# Autodesk Inventor assembly: LS Conveyor Axle
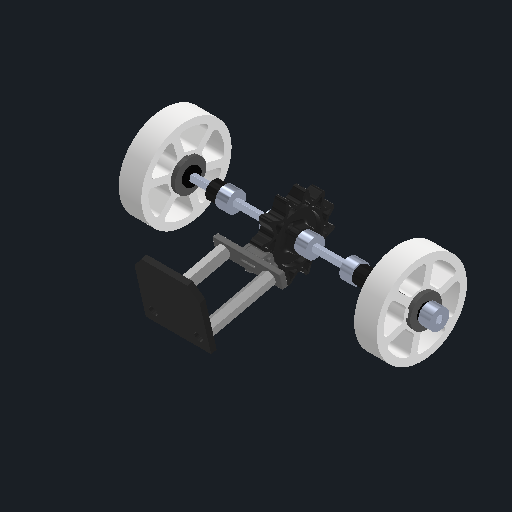
[picture p0: Inventor's stored thumbnail of the model, 512x512]
Saved by Autodesk Inventor 2025 (Build 290162000, 162)
## iProperties
Created: 2024-12-19
Part Number: LS Conveyor Axle
Document SubType Name: Assembly
Designer: Juan
Author: Juan
## Documents named in this file (14)
- C:\Users\Juan\Documents\GitHub\ATUM-VRC-High-Stakes-CAD\Protobot\LS Conveyor Axle.iam
- C:\Users\Juan\Documents\GitHub\ATUM-VRC-High-Stakes-CAD\VEX-CAD-Inventor\Motion\Sprockets\9P Sprocket\9P 12T Sprocket, Square.iam
- C:\Users\Juan\Documents\GitHub\ATUM-VRC-High-Stakes-CAD\VEX-CAD-Inventor\Motion\Sprockets\9P Sprocket.iam
- C:\Users\Juan\Documents\GitHub\ATUM-VRC-High-Stakes-CAD\VEX-CAD-Inventor\Motion\Chain 9P\Chain Attachment Link.ipt
- C:\Users\Juan\Documents\GitHub\ATUM-VRC-High-Stakes-CAD\Hook.ipt
- C:\Users\Juan\Documents\GitHub\ATUM-VRC-High-Stakes-CAD\VEX-CAD-Inventor\Structure\Standoff\Standoff 1.50.ipt
- C:\Users\Juan\Documents\GitHub\ATUM-VRC-High-Stakes-CAD\VEX-CAD-Inventor\Structure\Standoff.ipt
- C:\Users\Juan\Documents\GitHub\ATUM-VRC-High-Stakes-CAD\VEX-CAD-Inventor\Motion\Shaft LS\Shaft LS\Shaft LS 6.5.ipt
- C:\Users\Juan\Documents\GitHub\ATUM-VRC-High-Stakes-CAD\VEX-CAD-Inventor\Motion\Shaft LS\Shaft LS.ipt
- C:\Users\Juan\Documents\GitHub\ATUM-VRC-High-Stakes-CAD\VEX-CAD-Inventor\Motion\Shaft LS\Shaft Collar Metal\Shaft Collar No Screw.ipt
- C:\Users\Juan\Documents\GitHub\ATUM-VRC-High-Stakes-CAD\VEX-CAD-Inventor\Motion\Spacers\Spacer Nylon .375 OD\NSpacer .375 OD x .250.ipt
- C:\Users\Juan\Documents\GitHub\ATUM-VRC-High-Stakes-CAD\VEX-CAD-Inventor\Motion\Spacers\Spacer Nylon .375 OD.ipt
- C:\Users\Juan\Documents\GitHub\ATUM-VRC-High-Stakes-CAD\VEX-CAD-Inventor\Motion\Insert Square.ipt
- C:\Users\Juan\Documents\GitHub\ATUM-VRC-High-Stakes-CAD\Protobot\2.0 Flex Wheel with Insert.iam
## Components (20 placed, 9 different names)
1. 9P 12T Sprocket, Square:1 [sub-assembly]
2. Chain Attachment Link:1
3. Hook:1
4. Standoff 1.50:1
5. Standoff 1.50:2
6. Shaft LS 6.5:1
7. Shaft Collar No Screw:1
8. Shaft Collar No Screw:2
9. NSpacer .375 OD x .250:1
10. NSpacer .375 OD x .250:2
11. Shaft Collar No Screw:3
12. Shaft Collar No Screw:4
13. Insert Square:1
14. Insert Square:2
15. Insert Square:3
16. Insert Square:4
17. Shaft Collar No Screw:5
18. Shaft Collar No Screw:6
19. 2.0 Flex Wheel with Insert:1 [sub-assembly]
20. 2.0 Flex Wheel with Insert:2 [sub-assembly]
## Relationships (45: Mate 37, Angle 6, Flush 2)
- [Mate]: 9P 12T Sprocket, Square:1 ↔ Chain Attachment Link:1
- [Mate] (-2.54 mm): 9P 12T Sprocket, Square:1 ↔ Chain Attachment Link:1
- [Mate]: Chain Attachment Link:1 ↔ Standoff 1.50:1
- [Mate]: Chain Attachment Link:1 ↔ Standoff 1.50:2
- [Mate]: Chain Attachment Link:1 ↔ Standoff 1.50:2
- [Mate] (0.1524 mm): 9P 12T Sprocket, Square:1 ↔ Chain Attachment Link:1
- [Mate]: Chain Attachment Link:1 ↔ Standoff 1.50:1
- [Mate]: Hook:1 ↔ Standoff 1.50:1
- [Mate]: Hook:1 ↔ Standoff 1.50:2
- [Mate]: Hook:1 ↔ Standoff 1.50:2
- [Mate]: 9P 12T Sprocket, Square:1 ↔ Shaft LS 6.5:1
- [Mate]: 9P 12T Sprocket, Square:1 ↔ Shaft LS 6.5:1
- [Mate]: 9P 12T Sprocket, Square:1 ↔ Shaft Collar No Screw:1
- [Mate]: 9P 12T Sprocket, Square:1 ↔ Shaft Collar No Screw:2
- [Mate]: NSpacer .375 OD x .250:1 ↔ Shaft Collar No Screw:3
- [Mate]: NSpacer .375 OD x .250:1 ↔ Shaft Collar No Screw:3
- [Angle] (0 deg): Shaft LS 6.5:1 ↔ Shaft Collar No Screw:1
- [Angle] (0 deg): Shaft LS 6.5:1 ↔ Shaft Collar No Screw:2
- [Angle] (0 deg): Shaft LS 6.5:1 ↔ Shaft Collar No Screw:3
- [Mate]: NSpacer .375 OD x .250:2 ↔ Shaft Collar No Screw:4
- [Angle] (0 deg): Shaft LS 6.5:1 ↔ Shaft Collar No Screw:4
- [Mate]: Insert Square:1 ↔ 2.0 Flex Wheel with Insert:1
- [Mate]: Insert Square:1 ↔ 2.0 Flex Wheel with Insert:1
- [Mate]: Insert Square:2 ↔ 2.0 Flex Wheel with Insert:1
- [Mate]: Insert Square:2 ↔ 2.0 Flex Wheel with Insert:1
- [Mate]: Insert Square:3 ↔ 2.0 Flex Wheel with Insert:2
- [Mate]: Insert Square:3 ↔ 2.0 Flex Wheel with Insert:2
- [Mate]: Insert Square:4 ↔ 2.0 Flex Wheel with Insert:2
- [Mate]: Insert Square:4 ↔ 2.0 Flex Wheel with Insert:2
- [Mate]: Insert Square:3 ↔ 2.0 Flex Wheel with Insert:2
- [Mate]: Insert Square:4 ↔ 2.0 Flex Wheel with Insert:2
- [Mate]: Insert Square:1 ↔ 2.0 Flex Wheel with Insert:1
- [Mate]: Insert Square:2 ↔ 2.0 Flex Wheel with Insert:1
- [Mate]: Shaft LS 6.5:1 ↔ Insert Square:1
- [Mate]: Shaft LS 6.5:1 ↔ Insert Square:1
- [Mate]: Shaft LS 6.5:1 ↔ Insert Square:4
- [Mate]: Shaft LS 6.5:1 ↔ Insert Square:4
- [Mate]: Insert Square:1 ↔ Shaft Collar No Screw:5
- [Angle] (0 deg): Shaft LS 6.5:1 ↔ Shaft Collar No Screw:5
- [Mate]: Insert Square:4 ↔ Shaft Collar No Screw:6
- [Angle] (0 deg): Shaft LS 6.5:1 ↔ Shaft Collar No Screw:6
- [Mate]: Insert Square:4 ↔ Shaft Collar No Screw:6
- [Mate]: Insert Square:1 ↔ Shaft Collar No Screw:5
- [Flush]: Shaft LS 6.5:1 ↔ Shaft Collar No Screw:6
- [Flush]: Shaft LS 6.5:1 ↔ Shaft Collar No Screw:5
## Named parameters: d1540_d1536 = 0 mm, d1541_d1537 = 0 mm, d1542_d1538 = 0 mm, d1543_d1539 = 0 mm
